# Autodesk Inventor assembly: Slate TR1 Figurine
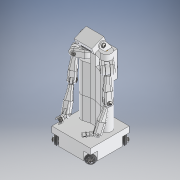
[picture p0: Inventor's stored thumbnail of the model, 180x180]
Saved by Autodesk Inventor 2017 SP1 (Build 210196100, 196)
## iProperties
Created: 2018-02-11
Part Number: Slate TR1 Figurine
Document SubType Name: Assembly
Designer: Zach
Author: Zach
## Documents named in this file (19)
- C:\Users\Zach\Documents\GitHub\tr1-figurine\Slate TR1 Figurine.iam
- C:\Users\Zach\Documents\GitHub\tr1-figurine\Base.ipt
- C:\Users\Zach\Documents\GitHub\tr1-figurine\Wheel.ipt
- C:\Users\Zach\Documents\Inventor\Content Center Files\R2017\en-US\SFS 2976\SFS 2976 - M3 x 12.ipt
- C:\Users\Zach\Documents\GitHub\tr1-figurine\Brass Bar - 3mm x 75mm.ipt
- C:\Users\Zach\Documents\GitHub\tr1-figurine\Body.ipt
- C:\Users\Zach\Documents\GitHub\tr1-figurine\Body2.ipt
- C:\Users\Zach\Documents\GitHub\tr1-figurine\Neck.ipt
- C:\Users\Zach\Documents\GitHub\tr1-figurine\Head.ipt
- C:\Users\Zach\Documents\GitHub\tr1-figurine\Backpack.ipt
- C:\Users\Zach\Documents\GitHub\tr1-figurine\Arm1.ipt
- C:\Users\Zach\Documents\GitHub\tr1-figurine\Arm2.ipt
- C:\Users\Zach\Documents\GitHub\tr1-figurine\Arm3.ipt
- C:\Users\Zach\Documents\GitHub\tr1-figurine\Arm4.ipt
- C:\Users\Zach\Documents\Inventor\Content Center Files\R2017\en-US\SFS 2976\SFS 2976 - M3 x 8.ipt
- C:\Users\Zach\Documents\GitHub\tr1-figurine\Arm5.ipt
- C:\Users\Zach\Documents\GitHub\tr1-figurine\Arm6.ipt
- C:\Users\Zach\Documents\GitHub\tr1-figurine\Arm7.ipt
- C:\Users\Zach\Documents\GitHub\tr1-figurine\Arm8.ipt
## Components (47 placed, 18 different names)
1. Base:1 — Mate:1, Mate:2, Mate:3, Mate:4, Mate:5, Mate:6, Mate:7, Mate:8, Mate:17, Mate:19, Mate:20, Mate:26, Mate:31, Mate:32, Mate:33
2. Backpack:1 — Mate:47, Mate:79, Mate:80, Mate:103, Mate:104, Mate:105, Mate:106
3. Body:1 — Mate:23, Mate:24, Mate:25, Mate:26, Mate:27, Mate:30, Mate:47, Mate:51, Mate:53, Mate:79, Mate:80, Angle:1
4. Body2:1 — Mate:27, Mate:30, Mate:34, Mate:35, Mate:36, Mate:37
5. Wheel:1 — Mate:1, Mate:2, Mate:9, Mate:10
6. Wheel:2 — Mate:3, Mate:4, Mate:11, Mate:12
7. Wheel:3 — Mate:5, Mate:6, Mate:15, Mate:16
8. Wheel:4 — Mate:7, Mate:8, Mate:13, Mate:14
9. Neck:1 — Mate:34, Mate:37, Mate:38, Mate:39, Mate:40, Mate:41, Mate:42, Mate:43, Mate:44, Mate:45, Angle:1
10. Head:1 — Mate:40, Mate:41
11. Arm1:1 — Mate:50, Mate:51, Mate:55, Mate:56, Mate:58, Mate:68, Mate:70
12. Arm1:2 — Mate:52, Mate:53, Mate:72, Mate:74, Mate:89, Mate:90, Mate:91, Mate:92
13. Arm2:1 — Mate:57, Mate:58, Mate:59, Mate:60, Mate:62
14. Arm2:2 — Mate:89, Mate:90
15. Arm3:1 — Mate:59, Mate:60, Mate:61, Mate:63, Mate:64, Mate:65, Mate:66
16. Arm3:2 — Mate:93, Mate:94
17. Arm4:1 — Mate:63, Mate:64, Mate:75, Mate:76
18. Arm4:2
19. Arm5:1 — Mate:67, Mate:68
20. Arm5:2 — Mate:69, Mate:70
21. Arm5:3 — Mate:71, Mate:72
22. Arm5:4 — Mate:73, Mate:74
23. Arm6:1 — Mate:75, Mate:76, Mate:77, Mate:78
24. Arm6:2
25. Arm7:1 — Mate:77, Mate:78, Mate:99, Mate:100
26. Arm7:2 — Mate:95, Mate:96
27. Arm8:1 — Mate:95, Mate:96, Mate:97, Mate:98
28. Arm8:2 — Mate:99, Mate:100, Mate:101, Mate:102
29. Brass Bar - 3mm x 75mm:1 — Mate:17, Mate:24, Mate:33, Mate:35, Mate:52, Mate:71, Mate:73
30. Brass Bar - 3mm x 75mm:2 — Mate:20, Mate:25, Mate:32
31. Brass Bar - 3mm x 75mm:3 — Mate:19, Mate:23, Mate:31, Mate:36, Mate:50, Mate:67, Mate:69
32. SFS 2976 M3 x 8:1 — Mate:65, Mate:66
33. SFS 2976 M3 x 8:2 — Mate:93, Mate:94
34. SFS 2976 M3 x 8:3 — Mate:97, Mate:98
35. SFS 2976 M3 x 8:4 — Mate:101, Mate:102
36. SFS 2976 M3 x 12:1 — Mate:9, Mate:10
37. SFS 2976 M3 x 12:2 — Mate:11, Mate:12
38. SFS 2976 M3 x 12:3 — Mate:13, Mate:14
39. SFS 2976 M3 x 12:4 — Mate:15, Mate:16
40. SFS 2976 M3 x 12:5 — Mate:38, Mate:39
41. SFS 2976 M3 x 12:6 — Mate:42, Mate:43
42. SFS 2976 M3 x 12:7 — Mate:44, Mate:45
43. SFS 2976 M3 x 12:9 — Mate:55, Mate:56, Mate:57
44. SFS 2976 M3 x 12:10 — Mate:61, Mate:62
45. SFS 2976 M3 x 12:11 — Mate:91, Mate:92
46. SFS 2976 M3 x 12:12 — Mate:104, Mate:106
47. SFS 2976 M3 x 12:13 — Mate:103, Mate:105
## Relationships (98: Mate 97, Angle 1)
- Mate:1: Base:1 ↔ Wheel:1
- Mate:2: Base:1 ↔ Wheel:1
- Mate:3: Base:1 ↔ Wheel:2
- Mate:4: Base:1 ↔ Wheel:2
- Mate:5: Base:1 ↔ Wheel:3
- Mate:6: Base:1 ↔ Wheel:3
- Mate:7: Base:1 ↔ Wheel:4
- Mate:8: Base:1 ↔ Wheel:4
- Mate:9: Wheel:1 ↔ SFS 2976 M3 x 12:1
- Mate:10: Wheel:1 ↔ SFS 2976 M3 x 12:1
- Mate:11: Wheel:2 ↔ SFS 2976 M3 x 12:2
- Mate:12: Wheel:2 ↔ SFS 2976 M3 x 12:2
- Mate:13: Wheel:4 ↔ SFS 2976 M3 x 12:3
- Mate:14: Wheel:4 ↔ SFS 2976 M3 x 12:3
- Mate:15: Wheel:3 ↔ SFS 2976 M3 x 12:4
- Mate:16: Wheel:3 ↔ SFS 2976 M3 x 12:4
- Mate:17: Base:1 ↔ Brass Bar - 3mm x 75mm:1
- Mate:19: Base:1 ↔ Brass Bar - 3mm x 75mm:3
- Mate:20: Base:1 ↔ Brass Bar - 3mm x 75mm:2
- Mate:23: Body:1 ↔ Brass Bar - 3mm x 75mm:3
- Mate:24: Body:1 ↔ Brass Bar - 3mm x 75mm:1
- Mate:25: Body:1 ↔ Brass Bar - 3mm x 75mm:2
- Mate:26: Base:1 ↔ Body:1
- Mate:27: Body:1 ↔ Body2:1
- Mate:30: Body:1 ↔ Body2:1
- Mate:31: Base:1 ↔ Brass Bar - 3mm x 75mm:3
- Mate:32: Base:1 ↔ Brass Bar - 3mm x 75mm:2
- Mate:33: Base:1 ↔ Brass Bar - 3mm x 75mm:1
- Mate:34: Body2:1 ↔ Neck:1
- Mate:35: Body2:1 ↔ Brass Bar - 3mm x 75mm:1
- Mate:36: Body2:1 ↔ Brass Bar - 3mm x 75mm:3
- Mate:37: Body2:1 ↔ Neck:1
- Mate:38: Neck:1 ↔ SFS 2976 M3 x 12:5
- Mate:39: Neck:1 ↔ SFS 2976 M3 x 12:5
- Mate:40: Neck:1 ↔ Head:1
- Mate:41 (0.25 mm): Neck:1 ↔ Head:1
- Mate:42: Neck:1 ↔ SFS 2976 M3 x 12:6
- Mate:43: Neck:1 ↔ SFS 2976 M3 x 12:6
- Mate:44: Neck:1 ↔ SFS 2976 M3 x 12:7
- Mate:45: Neck:1 ↔ SFS 2976 M3 x 12:7
- Mate:47: Backpack:1 ↔ Body:1
- Mate:50: Arm1:1 ↔ Brass Bar - 3mm x 75mm:3
- Mate:51 (2 mm): Body:1 ↔ Arm1:1
- Mate:52: Arm1:2 ↔ Brass Bar - 3mm x 75mm:1
- Mate:53 (2 mm): Body:1 ↔ Arm1:2
- Mate:55: Arm1:1 ↔ SFS 2976 M3 x 12:9
- Mate:56: Arm1:1 ↔ SFS 2976 M3 x 12:9
- Mate:57: Arm2:1 ↔ SFS 2976 M3 x 12:9
- Mate:58 (0.5 mm): Arm1:1 ↔ Arm2:1
- Mate:59: Arm2:1 ↔ Arm3:1
- Mate:60: Arm2:1 ↔ Arm3:1
- Mate:61: Arm3:1 ↔ SFS 2976 M3 x 12:10
- Mate:62: Arm2:1 ↔ SFS 2976 M3 x 12:10
- Mate:63: Arm3:1 ↔ Arm4:1
- Mate:64 (0.5 mm): Arm3:1 ↔ Arm4:1
- Mate:65: Arm3:1 ↔ SFS 2976 M3 x 8:1
- Mate:66: Arm3:1 ↔ SFS 2976 M3 x 8:1
- Mate:67: Arm5:1 ↔ Brass Bar - 3mm x 75mm:3
- Mate:68: Arm1:1 ↔ Arm5:1
- Mate:69: Arm5:2 ↔ Brass Bar - 3mm x 75mm:3
- Mate:70: Arm1:1 ↔ Arm5:2
- Mate:71: Arm5:3 ↔ Brass Bar - 3mm x 75mm:1
- Mate:72: Arm1:2 ↔ Arm5:3
- Mate:73: Arm5:4 ↔ Brass Bar - 3mm x 75mm:1
- Mate:74: Arm1:2 ↔ Arm5:4
- Mate:75: Arm4:1 ↔ Arm6:1
- Mate:76: Arm4:1 ↔ Arm6:1
- Mate:77: Arm6:1 ↔ Arm7:1
- Mate:78 (0.25 mm): Arm6:1 ↔ Arm7:1
- Mate:79: Backpack:1 ↔ Body:1
- Mate:80: Backpack:1 ↔ Body:1
- [Mate]: Arm2:2 ↔ Arm3:2
- [Mate]: Arm2:2 ↔ Arm3:2
- [Mate]: Arm3:2 ↔ Arm4:2
- [Mate] (0.5 mm): Arm3:2 ↔ Arm4:2
- [Mate]: Arm4:2 ↔ Arm6:2
- [Mate]: Arm4:2 ↔ Arm6:2
- [Mate]: Arm6:2 ↔ Arm7:2
- [Mate] (0.25 mm): Arm6:2 ↔ Arm7:2
- Mate:89 (0.5 mm): Arm1:2 ↔ Arm2:2
- Mate:90: Arm1:2 ↔ Arm2:2
- Mate:91: Arm1:2 ↔ SFS 2976 M3 x 12:11
- Mate:92: Arm1:2 ↔ SFS 2976 M3 x 12:11
- Mate:93: Arm3:2 ↔ SFS 2976 M3 x 8:2
- Mate:94: Arm3:2 ↔ SFS 2976 M3 x 8:2
- Angle:1 (0 deg): Body:1 ↔ Neck:1
- Mate:95: Arm7:2 ↔ Arm8:1
- Mate:96: Arm7:2 ↔ Arm8:1
- Mate:97: Arm8:1 ↔ SFS 2976 M3 x 8:3
- Mate:98: Arm8:1 ↔ SFS 2976 M3 x 8:3
- Mate:99: Arm7:1 ↔ Arm8:2
- Mate:100: Arm7:1 ↔ Arm8:2
- Mate:101: Arm8:2 ↔ SFS 2976 M3 x 8:4
- Mate:102: Arm8:2 ↔ SFS 2976 M3 x 8:4
- Mate:103: Backpack:1 ↔ SFS 2976 M3 x 12:13
- Mate:104: Backpack:1 ↔ SFS 2976 M3 x 12:12
- Mate:105: Backpack:1 ↔ SFS 2976 M3 x 12:13
- Mate:106: Backpack:1 ↔ SFS 2976 M3 x 12:12
## Named parameters: d80_d62 = 0 mm, d81_d63 = 0.5 mm, d82_d74 = 0 mm, d83_d75 = 0 mm, d84_d76 = 0 mm, d85_d77 = 0.25 mm, d86_d58 = 0 mm, d87_d59 = 0 mm
